# Autodesk Inventor assembly: highVoltageMppcBoard
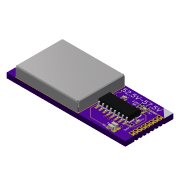
[picture p0: Inventor's stored thumbnail of the model, 180x180]
Saved by Autodesk Inventor 2016 SP2 (Build 200236200, 236)
## iProperties
Created: 2016-06-29
Part Number: highVoltageMppcBoard
Document SubType Name: Assembly
Designer: Jonathan
Author: Jonathan
## Documents named in this file (17)
- C:\Users\sawaiz\OneDrive\projects\mppcHighVoltage\cad\highVoltageMppcBoard.iam
- C:\Users\sawaiz\oneDrive\projects\mppcHighVoltage\cad\highVoltageMppcBoard.ipt
- C:\Users\sawaiz\oneDrive\projects\mppcHighVoltage\cad\electronics\qfn\qfn-12.ipt
- C:\Users\Jonathan\Documents\Projects\mppcHighVoltage\mppcHighVoltage\cad\electronics\qfn.ipt
- C:\Users\sawaiz\oneDrive\projects\mppcHighVoltage\cad\electronics\chipResistor\chipResistor-0402.ipt
- C:\Users\Jonathan\Documents\Projects\mppcHighVoltage\mppcHighVoltage\cad\electronics\chipResistor.ipt
- C:\Users\sawaiz\oneDrive\projects\mppcHighVoltage\cad\electronics\SOT23-3.ipt
- C:\Users\sawaiz\oneDrive\projects\mppcHighVoltage\cad\electronics\capacitor-1206.ipt
- C:\Users\Jonathan\Documents\Projects\mppcHighVoltage\mppcHighVoltage\cad\electronics\capacitor.ipt
- C:\Users\sawaiz\oneDrive\projects\mppcHighVoltage\cad\electronics\sod-80.ipt
- C:\Users\sawaiz\oneDrive\projects\mppcHighVoltage\cad\electronics\capacitor-0402.ipt
- C:\Users\sawaiz\oneDrive\projects\mppcHighVoltage\cad\electronics\SRN4018.ipt
- C:\Users\sawaiz\oneDrive\projects\mppcHighVoltage\cad\electronics\inductor-1007.ipt
- C:\Users\Jonathan\Documents\Projects\mppcHighVoltage\mppcHighVoltage\cad\electronics\inductor.ipt
- C:\Users\sawaiz\oneDrive\projects\mppcHighVoltage\cad\electronics\S02-20150300.ipt
- C:\Users\sawaiz\oneDrive\projects\mppcHighVoltage\cad\electronics\SOP-16.ipt
- C:\Users\sawaiz\oneDrive\projects\mppcHighVoltage\cad\electronics\capacitor-0603.ipt
## Components (27 placed, 12 different names)
1. highVoltageMppcBoard:1 — Angle:9, Angle:10, Angle:11, Angle:12, Angle:13, Angle:14, Flush:26, Angle:15, Mate:1, Mate:2, Tangent:1, Mate:3, Mate:4
2. qfn-12:1 — Flush:8, Angle:15, Mate:2
3. chipResistor-0402:1 — Flush:11, Flush:13, Flush:14
4. chipResistor-0402:2 — Flush:10, Flush:11, Flush:12, Flush:13
5. chipResistor-0402:3 — Flush:9, Flush:10, Flush:12
6. chipResistor-0402:4 — Flush:8, Flush:9
7. chipResistor-0402:5 — Flush:20, Flush:21
8. SOT23-3:1 — Flush:16, Flush:17
9. capacitor-1206:1 — Flush:21, Flush:22
10. capacitor-1206:2 — Flush:17, Flush:18
11. capacitor-1206:3 — Flush:18, Flush:19
12. capacitor-1206:4 — Flush:22
13. sod-80:1 — Tangent:1
14. capacitor-0402:5 — Flush:14, Flush:15
15. SRN4018:1 — Flush:15, Flush:16
16. inductor-1007:1 — Flush:19, Flush:20
17. S02-20150300:1 — Angle:9, Flush:26, Mate:1
18. SOP-16:1 — Mate:3
19. capacitor-0402:6 — Flush:29, Flush:31
20. capacitor-0603:7 — Flush:25, Angle:13, Flush:27, Flush:28
21. chipResistor-0402:6 — Flush:23, Flush:24, Angle:11
22. capacitor-0402:9 — Angle:10, Flush:33
23. chipResistor-0402:7 — Flush:23, Flush:28, Flush:29, Flush:30
24. chipResistor-0402:8 — Flush:24, Angle:12, Flush:33
25. capacitor-0603:10 — Flush:25, Angle:14, Flush:27, Flush:30, Mate:4
26. chipResistor-0402:9 — Flush:32
27. capacitor-0402:11 — Flush:31, Flush:32
## Relationships (53: Flush 33, Angle 15, Mate 4, Tangent 1)
- [Flush]: chipResistor-0402:1 ↔ chipResistor-0402:2
- [Flush]: chipResistor-0402:2 ↔ chipResistor-0402:3
- [Flush]: chipResistor-0402:3 ↔ chipResistor-0402:4
- [Flush]: chipResistor-0402:3 ↔ chipResistor-0402:5
- [Angle] (0 deg): chipResistor-0402:3 ↔ chipResistor-0402:4
- [Angle] (0 deg): chipResistor-0402:2 ↔ chipResistor-0402:3
- [Angle] (0 deg): chipResistor-0402:1 ↔ chipResistor-0402:2
- [Angle] (0 deg): chipResistor-0402:1 ↔ chipResistor-0402:5
- [Flush]: capacitor-1206:1 ↔ capacitor-1206:2
- [Flush]: capacitor-1206:1 ↔ capacitor-1206:3
- [Flush]: capacitor-1206:1 ↔ capacitor-1206:4
- [Angle] (0 deg): capacitor-1206:1 ↔ capacitor-1206:4
- [Angle] (0 deg): capacitor-1206:2 ↔ capacitor-1206:4
- [Angle] (0 deg): capacitor-1206:2 ↔ capacitor-1206:3
- [Angle] (0 deg): chipResistor-0402:1 ↔ capacitor-0402:5
- Flush:8: qfn-12:1 ↔ chipResistor-0402:4
- Flush:9: chipResistor-0402:3 ↔ chipResistor-0402:4
- Flush:10: chipResistor-0402:2 ↔ chipResistor-0402:3
- Flush:11: chipResistor-0402:1 ↔ chipResistor-0402:2
- Flush:12: chipResistor-0402:2 ↔ chipResistor-0402:3
- Flush:13: chipResistor-0402:1 ↔ chipResistor-0402:2
- Flush:14: chipResistor-0402:1 ↔ capacitor-0402:5
- Flush:15: capacitor-0402:5 ↔ SRN4018:1
- Flush:16: SOT23-3:1 ↔ SRN4018:1
- Flush:17: SOT23-3:1 ↔ capacitor-1206:2
- Flush:18: capacitor-1206:2 ↔ capacitor-1206:3
- Flush:19: capacitor-1206:3 ↔ inductor-1007:1
- Flush:20: chipResistor-0402:5 ↔ inductor-1007:1
- Flush:21: chipResistor-0402:5 ↔ capacitor-1206:1
- Flush:22: capacitor-1206:1 ↔ capacitor-1206:4
- Angle:9 (0 deg): highVoltageMppcBoard:1 ↔ S02-20150300:1
- Angle:10 (0 deg): highVoltageMppcBoard:1 ↔ capacitor-0402:9
- Flush:23: chipResistor-0402:6 ↔ chipResistor-0402:7
- Flush:24: chipResistor-0402:6 ↔ chipResistor-0402:8
- Angle:11 (0 deg): highVoltageMppcBoard:1 ↔ chipResistor-0402:6
- Angle:12 (0 deg): highVoltageMppcBoard:1 ↔ chipResistor-0402:8
- Flush:25: capacitor-0603:7 ↔ capacitor-0603:10
- Angle:13 (0 deg): highVoltageMppcBoard:1 ↔ capacitor-0603:7
- Angle:14 (0 deg): highVoltageMppcBoard:1 ↔ capacitor-0603:10
- Flush:26 (0.1 mm): highVoltageMppcBoard:1 ↔ S02-20150300:1
- Angle:15 (0 deg): highVoltageMppcBoard:1 ↔ qfn-12:1
- Mate:1: highVoltageMppcBoard:1 ↔ S02-20150300:1
- Mate:2: highVoltageMppcBoard:1 ↔ qfn-12:1
- Tangent:1: highVoltageMppcBoard:1 ↔ sod-80:1
- Mate:3: highVoltageMppcBoard:1 ↔ SOP-16:1
- Flush:27: capacitor-0603:7 ↔ capacitor-0603:10
- Flush:28: capacitor-0603:7 ↔ chipResistor-0402:7
- Flush:29: capacitor-0402:6 ↔ chipResistor-0402:7
- Flush:30: chipResistor-0402:7 ↔ capacitor-0603:10
- Flush:31: capacitor-0402:6 ↔ capacitor-0402:11
- Flush:32: chipResistor-0402:9 ↔ capacitor-0402:11
- Flush:33: capacitor-0402:9 ↔ chipResistor-0402:8
- Mate:4: highVoltageMppcBoard:1 ↔ capacitor-0603:10
